# Autodesk Inventor assembly: wheelR801
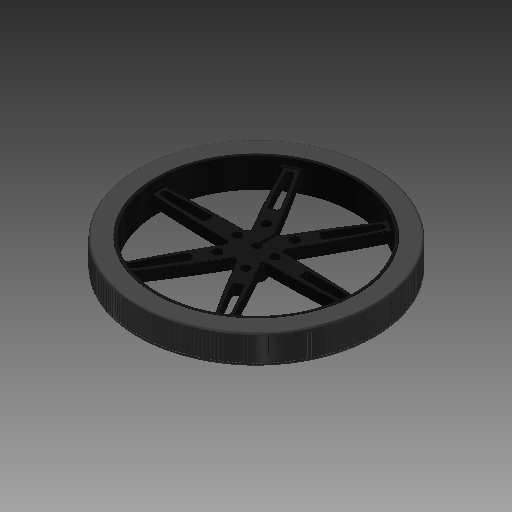
[picture p0: Inventor's stored thumbnail of the model, 512x512]
Saved by Autodesk Inventor 2018 (Build 220112000, 112)
## iProperties
Created: 2019-05-16
Part Number: wheelR801
Material: 一般
Document SubType Name: Assembly
Designer: ku_sk
Mass: 19.7 g
Surface Area: 203.81 cm^2
Volume: 18.5922 cm^3
Author: ku_sk
Sending System: Autodesk Inventor 2018
OS: Windows
FORMAT: text
GUISE: transmit
KEY: wheel
FILE: D:\windows\InventorProjects\Balboa32U4\parts\wheel.x_t
DATE: 2019-May-16 18:05:34
## Documents named in this file (3)
- D:\windows\InventorProjects\Balboa32U4\parts\wheel\wheelR801.iam
- D:\windows\InventorProjects\Balboa32U4\parts\wheel\parts\tyre1.ipt
- D:\windows\InventorProjects\Balboa32U4\parts\wheel\parts\wheel1.ipt
## Components (2 placed, 2 different names)
1. tyre1:1 — 角度:2, メイト:4, メイト:3
2. wheel1:1 — 角度:2, メイト:4, メイト:3, 角度:1, メイト:2, メイト:1
## Relationships (6: Mate 4, Angle 2)
- 角度:2 [Angle] (0 deg): tyre1:1 ↔ wheel1:1
- メイト:4 [Mate]: tyre1:1 ↔ wheel1:1
- メイト:3 [Mate]: tyre1:1 ↔ wheel1:1
- 角度:1 [Angle] (0 deg): wheel1:1
- メイト:2 [Mate]: wheel1:1
- メイト:1 [Mate]: wheel1:1
